# Autodesk Inventor assembly: Assembly2
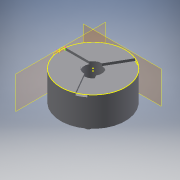
[picture p0: Inventor's stored thumbnail of the model, 180x180]
Saved by Autodesk Inventor 2016 (Build 200138000, 138)
## iProperties
Created: 2017-06-27
Part Number: Assembly2
Document SubType Name: Assembly
Designer: M228854
Author: M228854
## Documents named in this file (3)
- C:\Users\M228854\Downloads\Chucks\Assembly2.iam
- C:\Users\M228854\Downloads\Chucks\3 jaww.ipt
- C:\Users\M228854\Downloads\Chucks\rod.ipt
## Components (4 placed, 2 different names)
1. 3 jaww:1 — Mate:1, Mate:2, Mate:3
2. rod:1 — Mate:1
3. rod:2 — Mate:2
4. rod:3 — Mate:3
## Relationships (3: Mate 3)
- Mate:1: 3 jaww:1 ↔ rod:1
- Mate:2: 3 jaww:1 ↔ rod:2
- Mate:3: 3 jaww:1 ↔ rod:3
